# Autodesk Inventor assembly: commutator_assembly
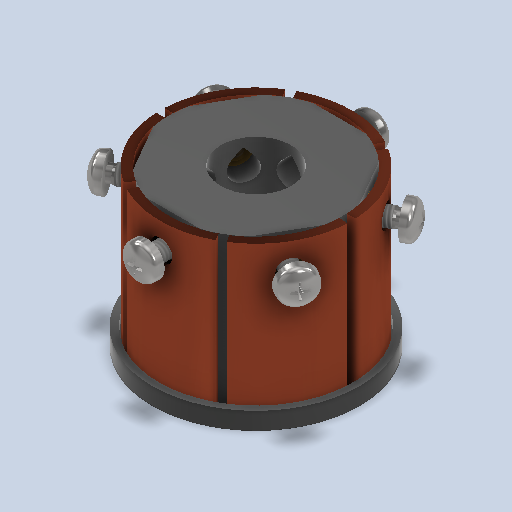
[picture p0: Inventor's stored thumbnail of the model, 512x512]
Saved by Autodesk Inventor 2025 (Build 290162000, 162)
## iProperties
Created: 2026-08-07
Part Number: commutator_assembly
Document SubType Name: Assembly
Designer: zzapa
Author: zzapa
## Documents named in this file (5)
- C:\Users\zzapa\Desktop\Projekty\elektronika\engine-project\model\assemblies\commutator_assembly.iam
- C:\Users\zzapa\Desktop\Projekty\elektronika\engine-project\model\parts\commutator_plastic.ipt
- C:\Users\zzapa\Desktop\Projekty\elektronika\engine-project\model\parts\commutator_plate.ipt
- C:\Users\zzapa\Documents\Inventor\Content Center Files\R2025\pl-PL\GB 809-88 A\Nut GB 809 A M2 x 3.ipt
- C:\Users\zzapa\Documents\Inventor\Content Center Files\R2025\pl-PL\BS EN ISO 7045 H\EN ISO 7045 - M2 x 4 - 4.8 - H(1).ipt
## Components (19 placed, 4 different names)
1. Nut GB/T 809-1988 Type A M2x3:1 — Zestawiające:5, Równoległe:2, Kątowe:8
2. Nut GB/T 809-1988 Type A M2x3:2 — Zestawiające:6, Równoległe:3, Zestawiające:10, Kątowe:7
3. Nut GB/T 809-1988 Type A M2x3:3 — Zestawiające:9, Równoległe:4, Kątowe:5
4. Nut GB/T 809-1988 Type A M2x3:4 — Zestawiające:8, Równoległe:5, Kątowe:6
5. Nut GB/T 809-1988 Type A M2x3:5 — Zestawiające:7, Równoległe:6, Kątowe:4
6. Nut GB/T 809-1988 Type A M2x3:6 — Zestawiające:4, Równoległe:7, Kątowe:3
7. BS EN ISO 7045 H - Metryczny M2 x 4 - 4.8 - H:1 — Zestawiające:10, Zestawiające:19, Kątowe:14
8. BS EN ISO 7045 H - Metryczny M2 x 4 - 4.8 - H:2 — Zestawiające:12, Zestawiające:18, Kątowe:12
9. BS EN ISO 7045 H - Metryczny M2 x 4 - 4.8 - H:3 — Zestawiające:15, Zestawiające:17, Kątowe:13
10. BS EN ISO 7045 H - Metryczny M2 x 4 - 4.8 - H:4 — Zestawiające:13, Zestawiające:21, Kątowe:11
11. BS EN ISO 7045 H - Metryczny M2 x 4 - 4.8 - H:5 — Zestawiające:11, Zestawiające:20, Kątowe:10
12. BS EN ISO 7045 H - Metryczny M2 x 4 - 4.8 - H:6 — Zestawiające:14, Zestawiające:16, Kątowe:9
13. commutator_plastic:1 — Zestawiające:1, Zestawiające:3, Kątowe:1, Kątowe:2, Równoległe:1, Zestawiające:4, Zestawiające:5, Zestawiające:6, Zestawiające:7, Zestawiające:8, Zestawiające:9, Równoległe:2, Równoległe:3, Równoległe:4, Równoległe:5, Równoległe:6, Równoległe:7, Zestawiające:16, Zestawiające:17, Zestawiające:18, Zestawiające:19, Zestawiające:20, Zestawiające:21, Zestawiające:22, Kątowe:3, Kątowe:4, Kątowe:5, Kątowe:6, Kątowe:7, Kątowe:8
14. commutator_plate:1 — Zestawiające:3, Kątowe:1, Równoległe:1, Zestawiające:14
15. commutator_plate:2 — Zestawiające:15
16. commutator_plate:3 — Zestawiające:12
17. commutator_plate:4
18. commutator_plate:5 — Zestawiające:11
19. commutator_plate:6 — Zestawiające:13
## Component patterns: (6 elements, first: commutator_plate:1)
## Relationships (42: Mate 21, Angle 14, Flush 7)
- Zestawiające:1 [Mate]: commutator_plastic:1
- Zestawiające:3 [Mate]: commutator_plastic:1 ↔ commutator_plate:1
- Kątowe:1 [Angle] (0 deg): commutator_plastic:1 ↔ commutator_plate:1
- Kątowe:2 [Angle] (0 deg): commutator_plastic:1
- Równoległe:1 [Flush]: commutator_plastic:1 ↔ commutator_plate:1
- Zestawiające:4 [Mate]: Nut GB/T 809-1988 Type A M2x3:6 ↔ commutator_plastic:1
- Zestawiające:5 [Mate]: Nut GB/T 809-1988 Type A M2x3:1 ↔ commutator_plastic:1
- Zestawiające:6 [Mate]: Nut GB/T 809-1988 Type A M2x3:2 ↔ commutator_plastic:1
- Zestawiające:7 [Mate]: Nut GB/T 809-1988 Type A M2x3:5 ↔ commutator_plastic:1
- Zestawiające:8 [Mate]: Nut GB/T 809-1988 Type A M2x3:4 ↔ commutator_plastic:1
- Zestawiające:9 [Mate]: Nut GB/T 809-1988 Type A M2x3:3 ↔ commutator_plastic:1
- Równoległe:2 [Flush]: Nut GB/T 809-1988 Type A M2x3:1 ↔ commutator_plastic:1
- Równoległe:3 [Flush]: Nut GB/T 809-1988 Type A M2x3:2 ↔ commutator_plastic:1
- Równoległe:4 [Flush]: Nut GB/T 809-1988 Type A M2x3:3 ↔ commutator_plastic:1
- Równoległe:5 [Flush]: Nut GB/T 809-1988 Type A M2x3:4 ↔ commutator_plastic:1
- Równoległe:6 [Flush]: Nut GB/T 809-1988 Type A M2x3:5 ↔ commutator_plastic:1
- Równoległe:7 [Flush]: Nut GB/T 809-1988 Type A M2x3:6 ↔ commutator_plastic:1
- Zestawiające:10 [Mate]: Nut GB/T 809-1988 Type A M2x3:2 ↔ BS EN ISO 7045 H - Metryczny M2 x 4 - 4.8 - H:1
- Zestawiające:11 [Mate]: BS EN ISO 7045 H - Metryczny M2 x 4 - 4.8 - H:5 ↔ commutator_plate:5
- Zestawiające:12 [Mate]: BS EN ISO 7045 H - Metryczny M2 x 4 - 4.8 - H:2 ↔ commutator_plate:3
- Zestawiające:13 [Mate]: BS EN ISO 7045 H - Metryczny M2 x 4 - 4.8 - H:4 ↔ commutator_plate:6
- Zestawiające:14 [Mate]: BS EN ISO 7045 H - Metryczny M2 x 4 - 4.8 - H:6 ↔ commutator_plate:1
- Zestawiające:15 [Mate]: BS EN ISO 7045 H - Metryczny M2 x 4 - 4.8 - H:3 ↔ commutator_plate:2
- Zestawiające:16 [Mate] (3 mm): BS EN ISO 7045 H - Metryczny M2 x 4 - 4.8 - H:6 ↔ commutator_plastic:1
- Zestawiające:17 [Mate] (3 mm): BS EN ISO 7045 H - Metryczny M2 x 4 - 4.8 - H:3 ↔ commutator_plastic:1
- Zestawiające:18 [Mate] (3 mm): BS EN ISO 7045 H - Metryczny M2 x 4 - 4.8 - H:2 ↔ commutator_plastic:1
- Zestawiające:19 [Mate] (3 mm): BS EN ISO 7045 H - Metryczny M2 x 4 - 4.8 - H:1 ↔ commutator_plastic:1
- Zestawiające:20 [Mate] (3 mm): BS EN ISO 7045 H - Metryczny M2 x 4 - 4.8 - H:5 ↔ commutator_plastic:1
- Zestawiające:21 [Mate] (3 mm): BS EN ISO 7045 H - Metryczny M2 x 4 - 4.8 - H:4 ↔ commutator_plastic:1
- Zestawiające:22 [Mate]: commutator_plastic:1
- Kątowe:3 [Angle] (0 deg): Nut GB/T 809-1988 Type A M2x3:6 ↔ commutator_plastic:1
- Kątowe:4 [Angle] (0 deg): Nut GB/T 809-1988 Type A M2x3:5 ↔ commutator_plastic:1
- Kątowe:5 [Angle] (0 deg): Nut GB/T 809-1988 Type A M2x3:3 ↔ commutator_plastic:1
- Kątowe:6 [Angle] (0 deg): Nut GB/T 809-1988 Type A M2x3:4 ↔ commutator_plastic:1
- Kątowe:7 [Angle] (0 deg): Nut GB/T 809-1988 Type A M2x3:2 ↔ commutator_plastic:1
- Kątowe:8 [Angle] (0 deg): Nut GB/T 809-1988 Type A M2x3:1 ↔ commutator_plastic:1
- Kątowe:9 [Angle] (0 deg): BS EN ISO 7045 H - Metryczny M2 x 4 - 4.8 - H:6
- Kątowe:10 [Angle] (0 deg): BS EN ISO 7045 H - Metryczny M2 x 4 - 4.8 - H:5
- Kątowe:11 [Angle] (0 deg): BS EN ISO 7045 H - Metryczny M2 x 4 - 4.8 - H:4
- Kątowe:12 [Angle] (0 deg): BS EN ISO 7045 H - Metryczny M2 x 4 - 4.8 - H:2
- Kątowe:13 [Angle] (0 deg): BS EN ISO 7045 H - Metryczny M2 x 4 - 4.8 - H:3
- Kątowe:14 [Angle] (0 deg): BS EN ISO 7045 H - Metryczny M2 x 4 - 4.8 - H:1
